# Autodesk Inventor assembly: 3 Motor Gearbox
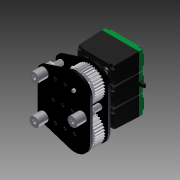
[picture p0: Inventor's stored thumbnail of the model, 180x180]
Saved by Autodesk Inventor 2014 SP1 (Build 180222100, 222)
## iProperties
Created: 2013-10-10
Part Number: 3 Motor Gearbox
Document SubType Name: Assembly
Designer: RyanHughes
Author: Andrew
Title: E:\My Documents\Inventor\VEX Robots\Sack Attack\15 defense\3 Motor Gearbox.stp
Creation Date: 2013-01-16
Sending System: Autodesk Inventor 2013
Preprocessor: Autodesk Inventor 2013
Author: RyanHughes
## Documents named in this file (7)
- C:\Users\Ryan\Desktop\sw\toss up 2ed A bot\drivetrain\3 Motor Gearbox.iam
- C:\Users\Ryan\Desktop\sw\toss up 2ed A bot\drivetrain\NAR gearplate.ipt
- C:\Users\Ryan\Desktop\sw\lib\Super Sonic Sparks VEX CAD Library\Motors & Sensors\2-Wire Motor 393-Without Wire.iam
- C:\Users\Ryan\Desktop\sw\lib\Aperture VEX CAD Library\Hardware\6-32\6-32_.500.ipt
- C:\Users\Ryan\Desktop\sw\toss up 2ed A bot\drivetrain\gear for gearbox.iam
- C:\Users\Ryan\Desktop\sw\toss up 2ed A bot\drivetrain\spacer for gearbox.iam
- C:\Users\Ryan\Desktop\sw\lib\Aperture VEX CAD Library\Shaft\2 inch Shaft.ipt
## Components (19 placed, 6 different names)
1. 3 Motor Gearbox:1 — Mate:2, Flush:1, Flush:2, Mate:25, Mate:26, Mate:27, Mate:28, Mate:29, Mate:30, Mate:37, Mate:45, Mate:46, Mate:47
2. 3 Motor Gearbox:2 — Flush:1, Flush:2, Mate:31, Mate:32, Mate:33, Mate:34, Mate:35, Mate:36
3. 396 motor:1 [sub-assembly] — Mate:41, Mate:42, Mate:43, Mate:44, Mate:45, Mate:46, Mate:47
4. 396 motor:2 [sub-assembly]
5. 396 motor:3 [sub-assembly] — Mate:1, Mate:2, Mate:3, Mate:38, Mate:39, Mate:40
6. 6-32_.500:1 — Mate:3
7. 6-32_.500:2
8. 6-32_.500:3
9. 6-32_.500:4 — Mate:1
10. 6-32_.500:5 — Mate:43
11. 6-32_.500:6 — Mate:44
12. gear for gearbox:1 [sub-assembly] — Mate:25, Mate:26
13. gear for gearbox:2 [sub-assembly] — Mate:27, Mate:28
14. gear for gearbox:3 [sub-assembly] — Mate:29, Mate:30
15. spacer for gearbox:1 [sub-assembly] — Mate:31, Mate:32, Mate:37
16. spacer for gearbox:2 [sub-assembly] — Mate:33, Mate:34
17. spacer for gearbox:3 [sub-assembly] — Mate:35, Mate:36
18. 2 inch Shaft:1 — Mate:38, Mate:39, Mate:40
19. 2 inch Shaft:2 — Mate:41, Mate:42
## Relationships (28: Mate 26, Flush 2)
- Mate:1: 396 motor:3 ↔ 6-32_.500:4
- Mate:2: 3 Motor Gearbox:1 ↔ 396 motor:3
- Mate:3: 396 motor:3 ↔ 6-32_.500:1
- Flush:1: 3 Motor Gearbox:1 ↔ 3 Motor Gearbox:2
- Flush:2: 3 Motor Gearbox:1 ↔ 3 Motor Gearbox:2
- Mate:25: 3 Motor Gearbox:1 ↔ gear for gearbox:1
- Mate:26: 3 Motor Gearbox:1 ↔ gear for gearbox:1
- Mate:27: 3 Motor Gearbox:1 ↔ gear for gearbox:2
- Mate:28: 3 Motor Gearbox:1 ↔ gear for gearbox:2
- Mate:29: 3 Motor Gearbox:1 ↔ gear for gearbox:3
- Mate:30: 3 Motor Gearbox:1 ↔ gear for gearbox:3
- Mate:31: 3 Motor Gearbox:2 ↔ spacer for gearbox:1
- Mate:32: 3 Motor Gearbox:2 ↔ spacer for gearbox:1
- Mate:33: 3 Motor Gearbox:2 ↔ spacer for gearbox:2
- Mate:34: 3 Motor Gearbox:2 ↔ spacer for gearbox:2
- Mate:35: 3 Motor Gearbox:2 ↔ spacer for gearbox:3
- Mate:36: 3 Motor Gearbox:2 ↔ spacer for gearbox:3
- Mate:37: 3 Motor Gearbox:1 ↔ spacer for gearbox:1
- Mate:38: 396 motor:3 ↔ 2 inch Shaft:1
- Mate:39: 396 motor:3 ↔ 2 inch Shaft:1
- Mate:40: 396 motor:3 ↔ 2 inch Shaft:1
- Mate:41: 396 motor:1 ↔ 2 inch Shaft:2
- Mate:42: 396 motor:1 ↔ 2 inch Shaft:2
- Mate:43: 396 motor:1 ↔ 6-32_.500:5
- Mate:44: 396 motor:1 ↔ 6-32_.500:6
- Mate:45: 3 Motor Gearbox:1 ↔ 396 motor:1
- Mate:46: 3 Motor Gearbox:1 ↔ 396 motor:1
- Mate:47: 3 Motor Gearbox:1 ↔ 396 motor:1
